# Autodesk Inventor assembly: smartrapcore
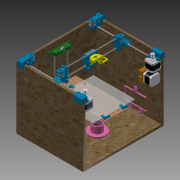
[picture p0: Inventor's stored thumbnail of the model, 180x180]
Saved by Autodesk Inventor 2015 (Build 190159000, 159)
## iProperties
Created: 2015-07-08
Part Number: smartrapcore
Document SubType Name: Assembly
Designer: hp
Author: hp
## Documents named in this file (32)
- D:\3D_Designs\Inventor\3D Printer\smartrapcore 2020\smartrapcore.iam
- D:\3D_Designs\Inventor\3D Printer\smartrapcore 2020\Parts\bottom_wall.ipt
- D:\3D_Designs\Inventor\3D Printer\smartrapcore 2020\Parts\side_wall.ipt
- D:\3D_Designs\Inventor\3D Printer\smartrapcore 2020\Parts\rear_wall.ipt
- D:\3D_Designs\Inventor\3D Printer\smartrapcore 2020\Parts\XYmotor_left.ipt
- D:\3D_Designs\Inventor\3D Printer\smartrapcore 2020\Parts\XYmotor_right.ipt
- D:\3D_Designs\Inventor\3D Printer\smartrapcore 2020\Parts\XYbearings_left.ipt
- D:\3D_Designs\Inventor\3D Printer\smartrapcore 2020\Parts\XYbearings_right.ipt
- D:\3D_Designs\Inventor\3D Printer\smartrapcore 2020\Parts\6mm_rod_265.ipt
- D:\3D_Designs\Inventor\3D Printer\smartrapcore 2020\Parts\Yslide_left.ipt
- D:\3D_Designs\Inventor\3D Printer\smartrapcore 2020\Parts\Yslide_right.ipt
- D:\3D_Designs\Inventor\3D Printer\smartrapcore 2020\Parts\head.ipt
- D:\3D_Designs\Inventor\3D Printer\smartrapcore 2020\Parts\LM6UU.ipt
- D:\3D_Designs\Inventor\3D Printer\smartrapcore 2020\Parts\jhead_adaptor.ipt
- D:\3D_Designs\Inventor\3D Printer\smartrapcore 2020\Parts\jhead_attach.ipt
- D:\3D_Designs\Inventor\3D Printer\smartrapcore 2020\Parts\NEMA_17_39mm.ipt
- D:\3D_Designs\Inventor\3D Printer\smartrapcore 2020\Parts\gt2-20t-6-5.ipt
- D:\3D_Designs\Inventor\3D Printer\smartrapcore 2020\Parts\Zbottom.ipt
- D:\3D_Designs\Inventor\3D Printer\smartrapcore 2020\Parts\8mm_rod_260.ipt
- D:\3D_Designs\Inventor\3D Printer\smartrapcore 2020\Parts\Ztop.ipt
- D:\3D_Designs\Inventor\3D Printer\smartrapcore 2020\Parts\Zslide.ipt
- D:\3D_Designs\Inventor\3D Printer\smartrapcore 2020\Parts\LM8UU.ipt
- D:\3D_Designs\Inventor\3D Printer\smartrapcore 2020\Parts\608ZZ.ipt
- D:\3D_Designs\Inventor\3D Printer\smartrapcore 2020\Parts\ramps_support.ipt
- D:\3D_Designs\Inventor\3D Printer\smartrapcore 2020\Parts\extruder_mk8_bottom.ipt
- D:\3D_Designs\Inventor\3D Printer\smartrapcore 2020\Parts\extruder_mk8_top.ipt
- D:\3D_Designs\Inventor\3D Printer\smartrapcore 2020\Parts\glass.ipt
- D:\3D_Designs\Inventor\3D Printer\smartrapcore 2020\Parts\bed support.ipt
- D:\3D_Designs\Inventor\3D Printer\smartrapcore 2020\Parts\glass clip.ipt
- D:\3D_Designs\Inventor\3D Printer\smartrapcore 2020\Parts\spoolholder46.ipt
- D:\3D_Designs\Inventor\3D Printer\smartrapcore 2020\Parts\fixalim.ipt
- D:\3D_Designs\Inventor\3D Printer\smartrapcore 2020\Parts\rubber cushion.ipt
## Components (65 placed, 31 different names)
1. bottom_wall:1 — Mate:1, Mate:2, Flush:1, Flush:2, Flush:3, Flush:4, Mate:3, Flush:5, Mate:59, Mate:95, Mate:120, Mate:121, Flush:32
2. side_wall:1 — Mate:1, Flush:1, Flush:2, Mate:4, Mate:5, Mate:6, Flush:6, Mate:9, Mate:10, Mate:122
3. side_wall:2 — Mate:2, Flush:3, Flush:4, Mate:8, Mate:12, Mate:14, Mate:15, Flush:7, Mate:61, Mate:94, Flush:27, Mate:104
4. rear_wall:1 — Mate:3, Mate:4, Flush:5, Mate:11, Mate:13, Mate:60
5. XYmotor_left:1 — Mate:5, Mate:6, Flush:6, Mate:45, Mate:46, Mate:48
6. XYmotor_right:1 — Mate:8, Mate:15, Flush:7, Mate:44, Mate:47, Mate:49
7. XYbearings_left:1 — Mate:9, Mate:10, Mate:11, Mate:16, Flush:9, Mate:71, Mate:72, Mate:73, Mate:74
8. XYbearings_right:1 — Mate:12, Mate:13, Mate:14, Mate:17, Flush:8, Mate:80, Mate:81, Mate:84, Mate:85
9. 6mm_rod_265:1 — Mate:16, Flush:9, Cylindrical:1
10. 6mm_rod_265:2 — Mate:17, Flush:8, Cylindrical:2
11. Yslide_left:1 — Mate:29, Mate:30, Flush:12, Mate:86, Mate:87, Mate:88, Mate:89, Mate:90, Mate:91, Flush:25
12. Yslide_right:1 — Mate:20, Mate:21, Mate:27, Mate:28, Flush:13, Flush:16, Mate:78, Mate:79, Mate:82, Mate:83
13. 6mm_rod_265:3 — Mate:20, Cylindrical:4, Mate:91, Flush:25, Mate:123
14. 6mm_rod_265:4 — Mate:21, Cylindrical:3, Mate:90
15. head:1 — Mate:33, Mate:34, Flush:14, Flush:15, Mate:35, Mate:36, Mate:37, Mate:38, Tangent:1, Mate:124
16. LM6UU:1 — Mate:26, Mate:27
17. LM6UU:2 — Mate:26, Mate:28, Flush:13, Cylindrical:2
18. LM6UU:3 — Mate:25, Mate:29
19. LM6UU:4 — Mate:25, Mate:30, Flush:12, Cylindrical:1
20. LM6UU:5 — Mate:35, Mate:123
21. LM6UU:6 — Mate:33, Flush:15
22. LM6UU:7 — Mate:36, Cylindrical:4, Tangent:1
23. LM6UU:8 — Mate:34, Flush:14, Cylindrical:3
24. jhead_adaptor:1 — Mate:37, Mate:38, Mate:107, Mate:108, Mate:109, Mate:124
25. jhead_attach:1 — Mate:107, Mate:108, Mate:109
26. NEMA_17_39mm:3 — Mate:44, Mate:47, Mate:49, Mate:51, Mate:105, Mate:106
27. NEMA_17_39mm:4 — Mate:45, Mate:46, Mate:48, Mate:50, Flush:26
28. gt2-20t-6-5:1 — Mate:50, Flush:26
29. gt2-20t-6-5:2 — Mate:51, Flush:16
30. Zbottom:1 — Mate:52, Mate:53, Flush:18, Flush:19, Mate:56, Mate:57, Mate:58, Mate:59, Mate:60, Mate:61
31. 8mm_rod_260:1 — Mate:52, Flush:18, Mate:54, Flush:20, Cylindrical:5
32. 8mm_rod_260:2 — Mate:53, Flush:19, Mate:55, Cylindrical:6
33. Ztop:1 — Mate:54, Mate:55, Flush:20, Mate:67, Mate:68
34. NEMA_17_39mm:5 — Mate:56, Mate:57, Mate:58, Mate:62, Flush:28
35. gt2-20t-6-5:3 — Mate:62, Flush:28
36. Zslide:1 — Mate:63, Mate:64, Mate:65, Mate:66, Flush:21, Flush:22, Flush:23, Flush:24, Mate:110, Mate:111, Mate:112
37. LM8UU:1 — Mate:63, Flush:21, Cylindrical:5
38. LM8UU:2 — Mate:65, Flush:23
39. LM8UU:3 — Mate:64, Flush:22, Cylindrical:6
40. LM8UU:4 — Mate:66, Flush:24
41. 608ZZ:1 — Mate:67, Mate:68
42. 608ZZ:4 — Mate:73, Mate:74
43. 608ZZ:5 — Mate:71, Mate:72
44. 608ZZ:6 — Mate:78, Mate:82
45. 608ZZ:7 — Mate:79, Mate:83
46. 608ZZ:8 — Mate:80, Mate:84
47. 608ZZ:9 — Mate:81, Mate:85
48. 608ZZ:10 — Mate:88, Mate:89
49. 608ZZ:11 — Mate:86, Mate:87
50. ramps_support:1 — Mate:94, Mate:95, Flush:27
51. extruder_mk8_bottom:1 — Mate:96, Mate:97, Mate:98, Mate:99, Mate:100, Mate:101, Mate:102, Mate:103, Mate:104, Mate:105
52. NEMA_17_39mm:6 — Mate:96, Mate:97, Mate:98, Mate:106
53. 608ZZ:12 — Mate:99, Mate:100
54. extruder_mk8_top:1 — Mate:101, Mate:102, Mate:103
55. bed support:1 — Mate:110, Mate:111, Mate:112, Mate:114, Mate:115, Mate:116, Mate:117, Mate:118, Mate:119, Mate:125, Mate:126, Mate:127, Mate:128, Flush:33, Flush:34
56. glass clip:1 — Mate:114, Mate:118
57. glass clip:2 — Mate:115, Mate:119
58. glass clip:3 — Mate:116, Mate:117
59. spoolholder46:1 — Mate:120
60. fixalim:1 — Mate:121, Mate:122, Flush:32
61. rubber cushion:1 — Mate:125, Mate:130
62. rubber cushion:2 — Mate:126
63. rubber cushion:3 — Mate:128
64. rubber cushion:4 — Mate:127, Mate:129
65. glass:1 — Mate:129, Mate:130, Flush:33, Flush:34
## Relationships (144: Mate 109, Flush 28, CylindricalJoint 6, Tangent 1)
- Mate:1: bottom_wall:1 ↔ side_wall:1
- Mate:2: bottom_wall:1 ↔ side_wall:2
- Flush:1: bottom_wall:1 ↔ side_wall:1
- Flush:2: bottom_wall:1 ↔ side_wall:1
- Flush:3: bottom_wall:1 ↔ side_wall:2
- Flush:4: bottom_wall:1 ↔ side_wall:2
- Mate:3: bottom_wall:1 ↔ rear_wall:1
- Mate:4: side_wall:1 ↔ rear_wall:1
- Flush:5: bottom_wall:1 ↔ rear_wall:1
- Mate:5: side_wall:1 ↔ XYmotor_left:1
- Mate:6: side_wall:1 ↔ XYmotor_left:1
- Flush:6: side_wall:1 ↔ XYmotor_left:1
- Mate:8: side_wall:2 ↔ XYmotor_right:1
- Mate:9: side_wall:1 ↔ XYbearings_left:1
- Mate:10: side_wall:1 ↔ XYbearings_left:1
- Mate:11: rear_wall:1 ↔ XYbearings_left:1
- Mate:12: side_wall:2 ↔ XYbearings_right:1
- Mate:13: rear_wall:1 ↔ XYbearings_right:1
- Mate:14: side_wall:2 ↔ XYbearings_right:1
- Mate:15: side_wall:2 ↔ XYmotor_right:1
- Flush:7: side_wall:2 ↔ XYmotor_right:1
- Mate:16: XYbearings_left:1 ↔ 6mm_rod_265:1
- Mate:17: XYbearings_right:1 ↔ 6mm_rod_265:2
- Flush:8: XYbearings_right:1 ↔ 6mm_rod_265:2
- Flush:9: XYbearings_left:1 ↔ 6mm_rod_265:1
- Mate:20: Yslide_right:1 ↔ 6mm_rod_265:3
- Mate:21: Yslide_right:1 ↔ 6mm_rod_265:4
- Mate:25: LM6UU:3 ↔ LM6UU:4
- Mate:26: LM6UU:1 ↔ LM6UU:2
- Mate:27: Yslide_right:1 ↔ LM6UU:1
- Mate:28: Yslide_right:1 ↔ LM6UU:2
- Mate:29: Yslide_left:1 ↔ LM6UU:3
- Mate:30: Yslide_left:1 ↔ LM6UU:4
- Flush:12 (-4 mm): Yslide_left:1 ↔ LM6UU:4
- Flush:13 (-4 mm): Yslide_right:1 ↔ LM6UU:2
- Cylindrical:1: 6mm_rod_265:1 ↔ LM6UU:4
- Cylindrical:2: 6mm_rod_265:2 ↔ LM6UU:2
- Mate:33: head:1 ↔ LM6UU:6
- Mate:34: head:1 ↔ LM6UU:8
- Flush:14: head:1 ↔ LM6UU:8
- Flush:15: head:1 ↔ LM6UU:6
- Mate:35: head:1 ↔ LM6UU:5
- Mate:36: head:1 ↔ LM6UU:7
- Cylindrical:3: 6mm_rod_265:4 ↔ LM6UU:8
- Cylindrical:4: 6mm_rod_265:3 ↔ LM6UU:7
- Mate:37: head:1 ↔ jhead_adaptor:1
- Mate:38 (1.1 mm): head:1 ↔ jhead_adaptor:1
- Mate:44: XYmotor_right:1 ↔ NEMA_17_39mm:3
- Mate:45: XYmotor_left:1 ↔ NEMA_17_39mm:4
- Mate:46: XYmotor_left:1 ↔ NEMA_17_39mm:4
- Mate:47: XYmotor_right:1 ↔ NEMA_17_39mm:3
- Mate:48: XYmotor_left:1 ↔ NEMA_17_39mm:4
- Mate:49: XYmotor_right:1 ↔ NEMA_17_39mm:3
- Mate:50: NEMA_17_39mm:4 ↔ gt2-20t-6-5:1
- Mate:51: NEMA_17_39mm:3 ↔ gt2-20t-6-5:2
- Flush:16: Yslide_right:1 ↔ gt2-20t-6-5:2
- Mate:52: Zbottom:1 ↔ 8mm_rod_260:1
- Mate:53: Zbottom:1 ↔ 8mm_rod_260:2
- Flush:18: Zbottom:1 ↔ 8mm_rod_260:1
- Flush:19: Zbottom:1 ↔ 8mm_rod_260:2
- Mate:54: 8mm_rod_260:1 ↔ Ztop:1
- Mate:55: 8mm_rod_260:2 ↔ Ztop:1
- Flush:20: 8mm_rod_260:1 ↔ Ztop:1
- Mate:56: Zbottom:1 ↔ NEMA_17_39mm:5
- Mate:57: Zbottom:1 ↔ NEMA_17_39mm:5
- Mate:58: Zbottom:1 ↔ NEMA_17_39mm:5
- Mate:59: bottom_wall:1 ↔ Zbottom:1
- Mate:60: rear_wall:1 ↔ Zbottom:1
- Mate:61 (132.5 mm): side_wall:2 ↔ Zbottom:1
- Mate:62: NEMA_17_39mm:5 ↔ gt2-20t-6-5:3
- Mate:63: Zslide:1 ↔ LM8UU:1
- Mate:64: Zslide:1 ↔ LM8UU:3
- Mate:65: Zslide:1 ↔ LM8UU:2
- Mate:66: Zslide:1 ↔ LM8UU:4
- Flush:21: Zslide:1 ↔ LM8UU:1
- Flush:22: Zslide:1 ↔ LM8UU:3
- Flush:23: Zslide:1 ↔ LM8UU:2
- Flush:24: Zslide:1 ↔ LM8UU:4
- Cylindrical:5: 8mm_rod_260:1 ↔ LM8UU:1
- Cylindrical:6: 8mm_rod_260:2 ↔ LM8UU:3
- Mate:67: Ztop:1 ↔ 608ZZ:1
- Mate:68: Ztop:1 ↔ 608ZZ:1
- Mate:71: XYbearings_left:1 ↔ 608ZZ:5
- Mate:72: XYbearings_left:1 ↔ 608ZZ:5
- Mate:73: XYbearings_left:1 ↔ 608ZZ:4
- Mate:74: XYbearings_left:1 ↔ 608ZZ:4
- Mate:78: Yslide_right:1 ↔ 608ZZ:6
- Mate:79: Yslide_right:1 ↔ 608ZZ:7
- Mate:80: XYbearings_right:1 ↔ 608ZZ:8
- Mate:81: XYbearings_right:1 ↔ 608ZZ:9
- Mate:82: Yslide_right:1 ↔ 608ZZ:6
- Mate:83: Yslide_right:1 ↔ 608ZZ:7
- Mate:84: XYbearings_right:1 ↔ 608ZZ:8
- Mate:85: XYbearings_right:1 ↔ 608ZZ:9
- Mate:86: Yslide_left:1 ↔ 608ZZ:11
- Mate:87: Yslide_left:1 ↔ 608ZZ:11
- Mate:88: Yslide_left:1 ↔ 608ZZ:10
- Mate:89: Yslide_left:1 ↔ 608ZZ:10
- Mate:90: Yslide_left:1 ↔ 6mm_rod_265:4
- Mate:91: Yslide_left:1 ↔ 6mm_rod_265:3
- Flush:25 (-1 mm): Yslide_left:1 ↔ 6mm_rod_265:3
- Flush:26 (23.7 mm): NEMA_17_39mm:4 ↔ gt2-20t-6-5:1
- Mate:94: side_wall:2 ↔ ramps_support:1
- Mate:95 (20 mm): bottom_wall:1 ↔ ramps_support:1
- Flush:27 (70 mm): side_wall:2 ↔ ramps_support:1
- Mate:96: extruder_mk8_bottom:1 ↔ NEMA_17_39mm:6
- Mate:97: extruder_mk8_bottom:1 ↔ NEMA_17_39mm:6
- Mate:98: extruder_mk8_bottom:1 ↔ NEMA_17_39mm:6
- Mate:99: extruder_mk8_bottom:1 ↔ 608ZZ:12
- Mate:100: extruder_mk8_bottom:1 ↔ 608ZZ:12
- Mate:101: extruder_mk8_bottom:1 ↔ extruder_mk8_top:1
- Mate:102: extruder_mk8_bottom:1 ↔ extruder_mk8_top:1
- Mate:103: extruder_mk8_bottom:1 ↔ extruder_mk8_top:1
- Mate:104: side_wall:2 ↔ extruder_mk8_bottom:1
- Mate:105: NEMA_17_39mm:3 ↔ extruder_mk8_bottom:1
- Mate:106 (15 mm): NEMA_17_39mm:3 ↔ NEMA_17_39mm:6
- Mate:107 (1 mm): jhead_adaptor:1 ↔ jhead_attach:1
- Mate:108: jhead_adaptor:1 ↔ jhead_attach:1
- Mate:109: jhead_adaptor:1 ↔ jhead_attach:1
- Flush:28 (-10.141 mm): NEMA_17_39mm:5 ↔ gt2-20t-6-5:3
- Mate:110: Zslide:1 ↔ bed support:1
- Mate:111: Zslide:1 ↔ bed support:1
- Mate:112: Zslide:1 ↔ bed support:1
- Mate:114: bed support:1 ↔ glass clip:1
- Mate:115: bed support:1 ↔ glass clip:2
- Mate:116: bed support:1 ↔ glass clip:3
- Mate:117: bed support:1 ↔ glass clip:3
- Mate:118: bed support:1 ↔ glass clip:1
- Mate:119: bed support:1 ↔ glass clip:2
- Mate:120: bottom_wall:1 ↔ spoolholder46:1
- Mate:121: bottom_wall:1 ↔ fixalim:1
- Mate:122: side_wall:1 ↔ fixalim:1
- Flush:32 (150 mm): bottom_wall:1 ↔ fixalim:1
- Mate:123: 6mm_rod_265:3 ↔ LM6UU:5
- Tangent:1 (0.1 mm): head:1 ↔ LM6UU:7
- Mate:124: head:1 ↔ jhead_adaptor:1
- Mate:125: bed support:1 ↔ rubber cushion:1
- Mate:126: bed support:1 ↔ rubber cushion:2
- Mate:127: bed support:1 ↔ rubber cushion:4
- Mate:128: bed support:1 ↔ rubber cushion:3
- Mate:129: rubber cushion:4 ↔ glass:1
- Mate:130: rubber cushion:1 ↔ glass:1
- Flush:33 (16 mm): bed support:1 ↔ glass:1
- Flush:34 (40 mm): bed support:1 ↔ glass:1
